# Autodesk Inventor assembly: 02_Baseplate
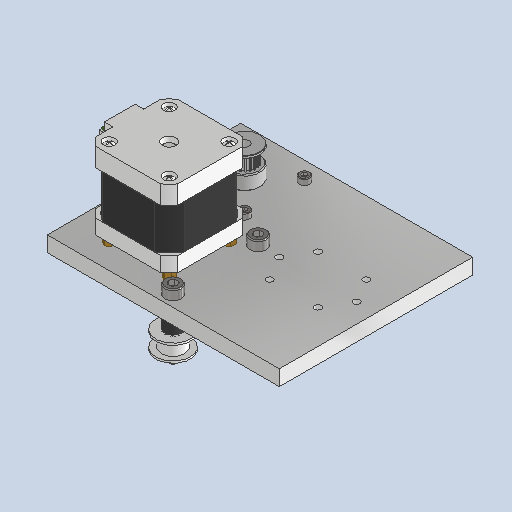
[picture p0: Inventor's stored thumbnail of the model, 512x512]
Saved by Autodesk Inventor 2022.2 (Build 262287010, 287A)
## iProperties
Created: 2022-05-03
Part Number: 02_Baseplate
Document SubType Name: Assembly
Designer: MXBD
Author: MXBD
## Documents named in this file (9)
- D:\Laser_Engraver\CAD\Assembly\02_Baseplate.iam
- D:\Laser_Engraver\CAD\Parts\14_XY_Plate.ipt
- D:\Laser_Engraver\CAD\Assemblies\UBG_Nema_17.iam
- D:\Laser_Engraver\CAD\Parts\11_GT2_Pulley_20_Teeth.ipt
- C:\Users\49152\Documents\Inventor\Content Center Files\R2022\de-DE\ISO 4762(2)\ISO 4762 - M3 x 12ISO.ipt
- C:\Users\49152\Documents\Inventor\Content Center Files\R2022\de-DE\ISO 4762(2)\ISO 4762 - M5 x 30ISO.ipt
- D:\Laser_Engraver\CAD\Parts\23_Spacers_7.7mm.ipt
- D:\Laser_Engraver\CAD\Parts\09_GT2_Idler_Pulley_Smooth.ipt
- C:\Users\49152\Documents\Inventor\Content Center Files\R2022\de-DE\DIN 439-2\DIN 439 - M5 x 0,8.ipt
## Components (21 placed, 8 different names)
1. 14_XY_Plate:1 — Passend:1, Passend:2, Passend:3, Passend:4, Winkel:1, Winkel:2, Passend:7, Passend:8, Passend:9, Passend:10, Passend:11, Passend:12, Passend:13, Passend:14, Passend:15, Passend:16, Passend:17, Passend:18, Passend:19, Passend:20, Passend:21, Passend:22, Passend:23, Passend:24, Passend:25, Passend:26, Passend:27, Passend:28, Passend:31, Passend:32
2. UBG_Nema_17:1 [sub-assembly] — Passend:1, Passend:4, Winkel:1, Passend:5
3. UBG_Nema_17:2 [sub-assembly] — Passend:2, Passend:3, Winkel:2, Passend:6
4. 11_GT2_Pulley_20_Teeth:1 — Passend:5, Passend:8
5. 11_GT2_Pulley_20_Teeth:2 — Passend:6, Passend:7
6. ISO 4762 M3 x 12:1 — Passend:10, Passend:18
7. ISO 4762 M3 x 12:2 — Passend:12, Passend:19
8. ISO 4762 M3 x 12:3 — Passend:9, Passend:17
9. ISO 4762 M3 x 12:4 — Passend:11, Passend:20
10. ISO 4762 M3 x 12:5 — Passend:14, Passend:23
11. ISO 4762 M3 x 12:6 — Passend:13, Passend:24
12. ISO 4762 M3 x 12:7 — Passend:15, Passend:22
13. ISO 4762 M3 x 12:8 — Passend:16, Passend:21
14. ISO 4762 M5 x 30:1 — Passend:25, Passend:27, Passend:29, Passend:33, Passend:37
15. ISO 4762 M5 x 30:2 — Passend:26, Passend:28, Passend:30, Passend:34, Passend:39
16. 23_Spacers_7.7mm:1 — Passend:29, Passend:31, Passend:35
17. 23_Spacers_7.7mm:2 — Passend:30, Passend:32, Passend:36
18. 09_GT2_Idler_Pulley_Smooth:1 — Passend:33, Passend:35, Passend:38
19. 09_GT2_Idler_Pulley_Smooth:2 — Passend:34, Passend:36, Passend:40
20. DIN 439-2 - ersetzt durch DIN EN 24035/28675 M5:1 — Passend:37, Passend:38
21. DIN 439-2 - ersetzt durch DIN EN 24035/28675 M5:2 — Passend:39, Passend:40
## Relationships (42: Mate 40, Angle 2)
- Passend:1 [Mate]: 14_XY_Plate:1 ↔ UBG_Nema_17:1
- Passend:2 [Mate]: 14_XY_Plate:1 ↔ UBG_Nema_17:2
- Passend:3 [Mate]: 14_XY_Plate:1 ↔ UBG_Nema_17:2
- Passend:4 [Mate]: 14_XY_Plate:1 ↔ UBG_Nema_17:1
- Winkel:1 [Angle] (0 deg): 14_XY_Plate:1 ↔ UBG_Nema_17:1
- Winkel:2 [Angle] (0 deg): 14_XY_Plate:1 ↔ UBG_Nema_17:2
- Passend:5 [Mate]: UBG_Nema_17:1 ↔ 11_GT2_Pulley_20_Teeth:1
- Passend:6 [Mate]: UBG_Nema_17:2 ↔ 11_GT2_Pulley_20_Teeth:2
- Passend:7 [Mate] (1 mm): 14_XY_Plate:1 ↔ 11_GT2_Pulley_20_Teeth:2
- Passend:8 [Mate] (1 mm): 14_XY_Plate:1 ↔ 11_GT2_Pulley_20_Teeth:1
- Passend:9 [Mate]: 14_XY_Plate:1 ↔ ISO 4762 M3 x 12:3
- Passend:10 [Mate]: 14_XY_Plate:1 ↔ ISO 4762 M3 x 12:1
- Passend:11 [Mate]: 14_XY_Plate:1 ↔ ISO 4762 M3 x 12:4
- Passend:12 [Mate]: 14_XY_Plate:1 ↔ ISO 4762 M3 x 12:2
- Passend:13 [Mate]: 14_XY_Plate:1 ↔ ISO 4762 M3 x 12:6
- Passend:14 [Mate]: 14_XY_Plate:1 ↔ ISO 4762 M3 x 12:5
- Passend:15 [Mate]: 14_XY_Plate:1 ↔ ISO 4762 M3 x 12:7
- Passend:16 [Mate]: 14_XY_Plate:1 ↔ ISO 4762 M3 x 12:8
- Passend:17 [Mate]: 14_XY_Plate:1 ↔ ISO 4762 M3 x 12:3
- Passend:18 [Mate]: 14_XY_Plate:1 ↔ ISO 4762 M3 x 12:1
- Passend:19 [Mate]: 14_XY_Plate:1 ↔ ISO 4762 M3 x 12:2
- Passend:20 [Mate]: 14_XY_Plate:1 ↔ ISO 4762 M3 x 12:4
- Passend:21 [Mate]: 14_XY_Plate:1 ↔ ISO 4762 M3 x 12:8
- Passend:22 [Mate]: 14_XY_Plate:1 ↔ ISO 4762 M3 x 12:7
- Passend:23 [Mate]: 14_XY_Plate:1 ↔ ISO 4762 M3 x 12:5
- Passend:24 [Mate]: 14_XY_Plate:1 ↔ ISO 4762 M3 x 12:6
- Passend:25 [Mate]: 14_XY_Plate:1 ↔ ISO 4762 M5 x 30:1
- Passend:26 [Mate]: 14_XY_Plate:1 ↔ ISO 4762 M5 x 30:2
- Passend:27 [Mate]: 14_XY_Plate:1 ↔ ISO 4762 M5 x 30:1
- Passend:28 [Mate]: 14_XY_Plate:1 ↔ ISO 4762 M5 x 30:2
- Passend:29 [Mate]: ISO 4762 M5 x 30:1 ↔ 23_Spacers_7.7mm:1
- Passend:30 [Mate]: ISO 4762 M5 x 30:2 ↔ 23_Spacers_7.7mm:2
- Passend:31 [Mate]: 14_XY_Plate:1 ↔ 23_Spacers_7.7mm:1
- Passend:32 [Mate]: 14_XY_Plate:1 ↔ 23_Spacers_7.7mm:2
- Passend:33 [Mate]: ISO 4762 M5 x 30:1 ↔ 09_GT2_Idler_Pulley_Smooth:1
- Passend:34 [Mate]: ISO 4762 M5 x 30:2 ↔ 09_GT2_Idler_Pulley_Smooth:2
- Passend:35 [Mate]: 23_Spacers_7.7mm:1 ↔ 09_GT2_Idler_Pulley_Smooth:1
- Passend:36 [Mate]: 23_Spacers_7.7mm:2 ↔ 09_GT2_Idler_Pulley_Smooth:2
- Passend:37 [Mate]: ISO 4762 M5 x 30:1 ↔ DIN 439-2 - ersetzt durch DIN EN 24035/28675 M5:1
- Passend:38 [Mate]: 09_GT2_Idler_Pulley_Smooth:1 ↔ DIN 439-2 - ersetzt durch DIN EN 24035/28675 M5:1
- Passend:39 [Mate]: ISO 4762 M5 x 30:2 ↔ DIN 439-2 - ersetzt durch DIN EN 24035/28675 M5:2
- Passend:40 [Mate]: 09_GT2_Idler_Pulley_Smooth:2 ↔ DIN 439-2 - ersetzt durch DIN EN 24035/28675 M5:2
